# Autodesk Inventor assembly: ElvMiddleFrame
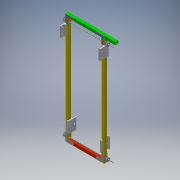
[picture p0: Inventor's stored thumbnail of the model, 180x180]
Saved by Autodesk Inventor 2019 (Build 230136000, 136)
## iProperties
Created: 2019-01-10
Part Number: ElvMiddleFrame
Document SubType Name: Assembly
Designer: james
Mass: 1353.41 g
Surface Area: 6550.04 cm^2
Volume: 725.529 cm^3
Density: 1.86541 g/cm^3
Author: james
## Documents named in this file (8)
- F:\JimsDesign\2019CHS4089\ElvMiddleFrame.iam
- F:\JimsDesign\2019CHS4089\ElvCrossBeam.ipt
- F:\JimsDesign\2019CHS4089\ElvMiddleBeam.ipt
- F:\JimsDesign\2019CHS4089\ElvShaft.iam
- F:\JimsDesign\2019CHS4089\ElvTopBeam.ipt
- F:\JimsDesign\2019CHS4089\elvRivetPlate.ipt
- F:\JimsDesign\2019CHS4089\ElvDelV5.ipt
- F:\JimsDesign\2019CHS4089\ElvDelV6.ipt
## Components (18 placed, 7 different names)
1. ElvCrossBeam:2 — Mate:25, Mate:26, Mate:27, Mate:28, Mate:29, Mate:30
2. ElvMiddleBeam:1 — Mate:31, Mate:32, Mate:33, Mate:43, Mate:49, Mate:50, Mate:53, Mate:54, Mate:55, Mate:59, Mate:60, Mate:61, Mate:65, Mate:66, Mate:67
3. ElvMiddleBeam:2 — Mate:3, Mate:5, Mate:21, Mate:23, Flush:9, Mate:24, Mate:34, Mate:35, Mate:36, Mate:46, Mate:51, Mate:52, Mate:56, Mate:57, Mate:58, Mate:68, Mate:69, Mate:70
4. ElvShaft:1 [sub-assembly] — Mate:5
5. ElvShaft:2 [sub-assembly] — Mate:3, Mate:21
6. ElvTopBeam:1 — Mate:37, Mate:38, Mate:39, Mate:40, Mate:41, Mate:42, Mate:62, Mate:63, Mate:64
7. elvRivetPlate:1 — Mate:23, Flush:9, Mate:24, Mate:25, Mate:26, Mate:27
8. elvRivetPlate:2 — Mate:28, Mate:29, Mate:30, Mate:31, Mate:32, Mate:33
9. elvRivetPlate:3 — Mate:34, Mate:35, Mate:36, Mate:37, Mate:38, Mate:39
10. elvRivetPlate:4 — Mate:40, Mate:41, Mate:42
11. ElvDelV5:1 — Mate:43, Mate:49, Mate:50
12. ElvDelV5:2 — Mate:46, Mate:51, Mate:52
13. elvRivetPlate:5 — Mate:53, Mate:54, Mate:55
14. elvRivetPlate:6 — Mate:56, Mate:57, Mate:58
15. elvRivetPlate:7 — Mate:59, Mate:60, Mate:61
16. elvRivetPlate:8 — Mate:62, Mate:63, Mate:64
17. ElvDelV6:1 — Mate:65, Mate:66, Mate:67
18. ElvDelV6:2 — Mate:68, Mate:69, Mate:70
## Relationships (48: Mate 47, Flush 1)
- Mate:3: ElvMiddleBeam:2 ↔ ElvShaft:2
- Mate:5: ElvMiddleBeam:2 ↔ ElvShaft:1
- Mate:21: ElvMiddleBeam:2 ↔ ElvShaft:2
- Mate:23: ElvMiddleBeam:2 ↔ elvRivetPlate:1
- Flush:9: ElvMiddleBeam:2 ↔ elvRivetPlate:1
- Mate:24: ElvMiddleBeam:2 ↔ elvRivetPlate:1
- Mate:25: ElvCrossBeam:2 ↔ elvRivetPlate:1
- Mate:26: ElvCrossBeam:2 ↔ elvRivetPlate:1
- Mate:27: ElvCrossBeam:2 ↔ elvRivetPlate:1
- Mate:28: ElvCrossBeam:2 ↔ elvRivetPlate:2
- Mate:29: ElvCrossBeam:2 ↔ elvRivetPlate:2
- Mate:30: ElvCrossBeam:2 ↔ elvRivetPlate:2
- Mate:31: ElvMiddleBeam:1 ↔ elvRivetPlate:2
- Mate:32: ElvMiddleBeam:1 ↔ elvRivetPlate:2
- Mate:33: ElvMiddleBeam:1 ↔ elvRivetPlate:2
- Mate:34: ElvMiddleBeam:2 ↔ elvRivetPlate:3
- Mate:35: ElvMiddleBeam:2 ↔ elvRivetPlate:3
- Mate:36: ElvMiddleBeam:2 ↔ elvRivetPlate:3
- Mate:37: ElvTopBeam:1 ↔ elvRivetPlate:3
- Mate:38: ElvTopBeam:1 ↔ elvRivetPlate:3
- Mate:39: ElvTopBeam:1 ↔ elvRivetPlate:3
- Mate:40: ElvTopBeam:1 ↔ elvRivetPlate:4
- Mate:41: ElvTopBeam:1 ↔ elvRivetPlate:4
- Mate:42: ElvTopBeam:1 ↔ elvRivetPlate:4
- Mate:43: ElvMiddleBeam:1 ↔ ElvDelV5:1
- Mate:46: ElvMiddleBeam:2 ↔ ElvDelV5:2
- Mate:49: ElvMiddleBeam:1 ↔ ElvDelV5:1
- Mate:50: ElvMiddleBeam:1 ↔ ElvDelV5:1
- Mate:51: ElvMiddleBeam:2 ↔ ElvDelV5:2
- Mate:52: ElvMiddleBeam:2 ↔ ElvDelV5:2
- Mate:53: ElvMiddleBeam:1 ↔ elvRivetPlate:5
- Mate:54: ElvMiddleBeam:1 ↔ elvRivetPlate:5
- Mate:55: ElvMiddleBeam:1 ↔ elvRivetPlate:5
- Mate:56: ElvMiddleBeam:2 ↔ elvRivetPlate:6
- Mate:57: ElvMiddleBeam:2 ↔ elvRivetPlate:6
- Mate:58: ElvMiddleBeam:2 ↔ elvRivetPlate:6
- Mate:59: ElvMiddleBeam:1 ↔ elvRivetPlate:7
- Mate:60: ElvMiddleBeam:1 ↔ elvRivetPlate:7
- Mate:61: ElvMiddleBeam:1 ↔ elvRivetPlate:7
- Mate:62: ElvTopBeam:1 ↔ elvRivetPlate:8
- Mate:63: ElvTopBeam:1 ↔ elvRivetPlate:8
- Mate:64: ElvTopBeam:1 ↔ elvRivetPlate:8
- Mate:65: ElvMiddleBeam:1 ↔ ElvDelV6:1
- Mate:66: ElvMiddleBeam:1 ↔ ElvDelV6:1
- Mate:67: ElvMiddleBeam:1 ↔ ElvDelV6:1
- Mate:68: ElvMiddleBeam:2 ↔ ElvDelV6:2
- Mate:69: ElvMiddleBeam:2 ↔ ElvDelV6:2
- Mate:70: ElvMiddleBeam:2 ↔ ElvDelV6:2
